# Autodesk Inventor assembly: Track Idler Assembly
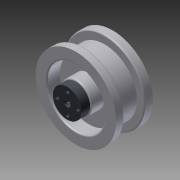
[picture p0: Inventor's stored thumbnail of the model, 180x180]
Saved by Autodesk Inventor 2015 (Build 190159000, 159)
## iProperties
Created: 2015-09-26
Part Number: Track Idler Assembly
Document SubType Name: Assembly
Designer: Jing-Chen
Author: Jing-Chen
## Documents named in this file (4)
- C:\Users\Jing-Chen\Desktop\Bionic Hybrids 2016\Bionic-Hybrids\CAD\Drivetrain\Sub-Assemblies\Track Idler Assembly.iam
- C:\Users\Jing-Chen\Desktop\Bionic Hybrids 2016\Bionic-Hybrids\Stock\Track Idler - 73646.ipt
- C:\Users\Jing-Chen\Desktop\Bionic Hybrids 2016\Bionic-Hybrids\Stock\Shaft Collar-Setscrew, Axle, Mountable - 739172.iam
- C:\Users\Jing-Chen\Desktop\Bionic Hybrids 2016\Bionic-Hybrids\Stock\Bearing-Thrust - 739091.ipt
## Components (3 placed, 3 different names)
1. Track Idler - 73646:1 — Mate:1, Mate:2, Mate:3, Mate:4, Mate:5
2. Shaft Collar-Setscrew, Axle, Mountable - 739172:1 [sub-assembly] — Mate:1, Mate:2, Mate:3
3. Bearing-Thrust - 739091:1 — Mate:4, Mate:5
## Relationships (5: Mate 5)
- Mate:1: Track Idler - 73646:1 ↔ Shaft Collar-Setscrew, Axle, Mountable - 739172:1
- Mate:2: Track Idler - 73646:1 ↔ Shaft Collar-Setscrew, Axle, Mountable - 739172:1
- Mate:3: Track Idler - 73646:1 ↔ Shaft Collar-Setscrew, Axle, Mountable - 739172:1
- Mate:4: Track Idler - 73646:1 ↔ Bearing-Thrust - 739091:1
- Mate:5: Track Idler - 73646:1 ↔ Bearing-Thrust - 739091:1
